# Autodesk Inventor assembly: fight_robot_fin2
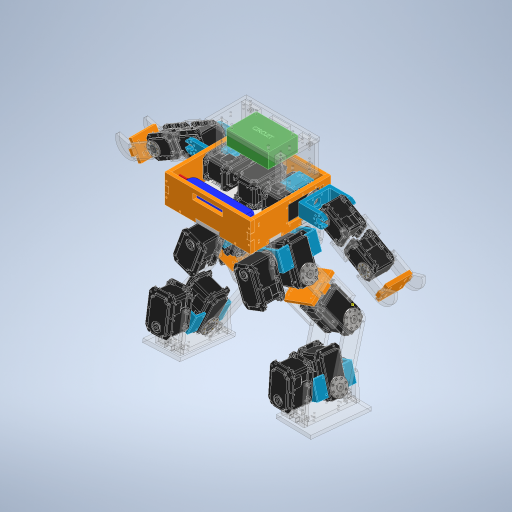
[picture p0: Inventor's stored thumbnail of the model, 512x512]
Saved by Autodesk Inventor 2024 (Build 280153000, 153)
## iProperties
Created: 2024-09-16
Part Number: fight_robot_fin2
Document SubType Name: Assembly
Designer: jmha0
Author: jmha0
## Documents named in this file (16)
- C:\Users\jmha0\OneDrive\바탕 화면\19th_intern_hjm_fight_robot\부품\fight_robot_fin2.iam
- C:\Users\jmha0\OneDrive\바탕 화면\19th_intern_hjm_fight_robot\부품\Lower_Body\waist\waist_fin1.iam
- C:\Users\jmha0\OneDrive\바탕 화면\19th_intern_hjm_fight_robot\부품\Lower_Body\pelvis_w_motor\pelvis_w_motor_fin1.iam
- C:\Users\jmha0\OneDrive\바탕 화면\19th_intern_hjm_fight_robot\부품\Lower_Body\pelvis_w_motor\pelvis_w_motor_fin1_opp.iam
- C:\Users\jmha0\OneDrive\바탕 화면\19th_intern_hjm_fight_robot\부품\Lower_Body\knee_w_motor\knee_fin1.iam
- C:\Users\jmha0\OneDrive\바탕 화면\19th_intern_hjm_fight_robot\부품\Lower_Body\ankle_w_feet\ankle_w_feet_right.iam
- C:\Users\jmha0\OneDrive\바탕 화면\19th_intern_hjm_fight_robot\부품\Lower_Body\ankle_w_feet\ankle_w_feet_left.iam
- C:\Users\jmha0\OneDrive\바탕 화면\19th_intern_hjm_fight_robot\부품\Upper_Body\etc\long_horn1.ipt
- C:\Users\jmha0\OneDrive\바탕 화면\19th_intern_hjm_fight_robot\부품\Upper_Body\Upper\upper_fin1.iam
- C:\Users\jmha0\OneDrive\바탕 화면\19th_intern_hjm_fight_robot\부품\Upper_Body\arm\arm_fin_left1.iam
- C:\Users\jmha0\OneDrive\바탕 화면\19th_intern_hjm_fight_robot\부품\Upper_Body\arm\arm_fin_right1.iam
- C:\Users\jmha0\OneDrive\바탕 화면\19th_intern_hjm_fight_robot\부품\Upper_Body\hand\hand_fin1_opp.iam
- C:\Users\jmha0\OneDrive\바탕 화면\19th_intern_hjm_fight_robot\부품\Upper_Body\hand\hand_fin1.iam
- C:\Users\jmha0\OneDrive\바탕 화면\19th_intern_hjm_fight_robot\부품\Upper_Body\head\head_fin1.iam
- C:\Users\jmha0\OneDrive\바탕 화면\19th_intern_hjm_fight_robot\부품\battery\Enrichpower_2200mAh_11.1V_30C.ipt
- C:\Users\jmha0\OneDrive\바탕 화면\19th_intern_hjm_fight_robot\부품\circuit\Circuit.ipt
## Components (16 placed, 15 different names)
1. waist_fin1:1 [sub-assembly] — 메이트:1, 각도:1, 메이트:2, 각도:2, 각도:3, 각도:4, 삽입:5, 삽입:6
2. pelvis_w_motor_fin1:1 [sub-assembly] — 메이트:2, 각도:2, 각도:3, 삽입:1, 삽입:2
3. pelvis_w_motor_fin1_opp:1 [sub-assembly] — 메이트:1, 각도:1, 각도:4, 삽입:3, 삽입:4
4. knee_fin1:1 [sub-assembly] — 삽입:3, 삽입:4, 메이트:3, 메이트:4
5. knee_fin1:2 [sub-assembly] — 삽입:1, 삽입:2, 메이트:5, 메이트:6
6. ankle_w_feet_right:1 [sub-assembly] — 메이트:3, 메이트:4
7. ankle_w_feet_left:1 [sub-assembly] — 메이트:5, 메이트:6
8. long_horn1:1 — 삽입:5, 삽입:6, 삽입:7, 삽입:8
9. upper_fin1:1 [sub-assembly] — 삽입:7, 삽입:8, 삽입:9, 삽입:10, 삽입:11, 삽입:12, 삽입:17, 삽입:18, 메이트:7, 메이트:8
10. arm_fin_left1:1 [sub-assembly] — 삽입:9, 삽입:10, 삽입:13, 삽입:14
11. arm_fin_right1:1 [sub-assembly] — 삽입:11, 삽입:12, 삽입:15, 삽입:16
12. hand_fin1_opp:1 [sub-assembly] — 삽입:15, 삽입:16
13. hand_fin1:1 [sub-assembly] — 삽입:13, 삽입:14
14. head_fin1:1 [sub-assembly] — 삽입:17, 삽입:18, 삽입:19, 삽입:20
15. Enrichpower_2200mAh_11.1V_30C:1 — 메이트:7, 메이트:8
16. Circuit:1 — 삽입:19, 삽입:20
## Relationships (32: Insert 20, Mate 8, Angle 4)
- 메이트:1 [Mate]: waist_fin1:1 ↔ pelvis_w_motor_fin1_opp:1
- 각도:1 [Angle] (0 deg): waist_fin1:1 ↔ pelvis_w_motor_fin1_opp:1
- 메이트:2 [Mate]: waist_fin1:1 ↔ pelvis_w_motor_fin1:1
- 각도:2 [Angle] (0 deg): waist_fin1:1 ↔ pelvis_w_motor_fin1:1
- 각도:3 [Angle] (-20 deg): waist_fin1:1 ↔ pelvis_w_motor_fin1:1
- 각도:4 [Angle] (20 deg): waist_fin1:1 ↔ pelvis_w_motor_fin1_opp:1
- 삽입:1 [Insert]: pelvis_w_motor_fin1:1 ↔ knee_fin1:2
- 삽입:2 [Insert]: pelvis_w_motor_fin1:1 ↔ knee_fin1:2
- 삽입:3 [Insert]: pelvis_w_motor_fin1_opp:1 ↔ knee_fin1:1
- 삽입:4 [Insert]: pelvis_w_motor_fin1_opp:1 ↔ knee_fin1:1
- 메이트:3 [Mate]: knee_fin1:1 ↔ ankle_w_feet_right:1
- 메이트:4 [Mate]: knee_fin1:1 ↔ ankle_w_feet_right:1
- 메이트:5 [Mate]: knee_fin1:2 ↔ ankle_w_feet_left:1
- 메이트:6 [Mate]: knee_fin1:2 ↔ ankle_w_feet_left:1
- 삽입:5 [Insert]: waist_fin1:1 ↔ long_horn1:1
- 삽입:6 [Insert]: waist_fin1:1 ↔ long_horn1:1
- 삽입:7 [Insert]: long_horn1:1 ↔ upper_fin1:1
- 삽입:8 [Insert]: long_horn1:1 ↔ upper_fin1:1
- 삽입:9 [Insert]: upper_fin1:1 ↔ arm_fin_left1:1
- 삽입:10 [Insert]: upper_fin1:1 ↔ arm_fin_left1:1
- 삽입:11 [Insert]: upper_fin1:1 ↔ arm_fin_right1:1
- 삽입:12 [Insert]: upper_fin1:1 ↔ arm_fin_right1:1
- 삽입:13 [Insert]: arm_fin_left1:1 ↔ hand_fin1:1
- 삽입:14 [Insert]: arm_fin_left1:1 ↔ hand_fin1:1
- 삽입:15 [Insert]: arm_fin_right1:1 ↔ hand_fin1_opp:1
- 삽입:16 [Insert]: arm_fin_right1:1 ↔ hand_fin1_opp:1
- 삽입:17 [Insert]: upper_fin1:1 ↔ head_fin1:1
- 삽입:18 [Insert]: upper_fin1:1 ↔ head_fin1:1
- 메이트:7 [Mate]: upper_fin1:1 ↔ Enrichpower_2200mAh_11.1V_30C:1
- 메이트:8 [Mate]: upper_fin1:1 ↔ Enrichpower_2200mAh_11.1V_30C:1
- 삽입:19 [Insert]: head_fin1:1 ↔ Circuit:1
- 삽입:20 [Insert]: head_fin1:1 ↔ Circuit:1
